# Autodesk Inventor assembly: Segment_Traeger_v1
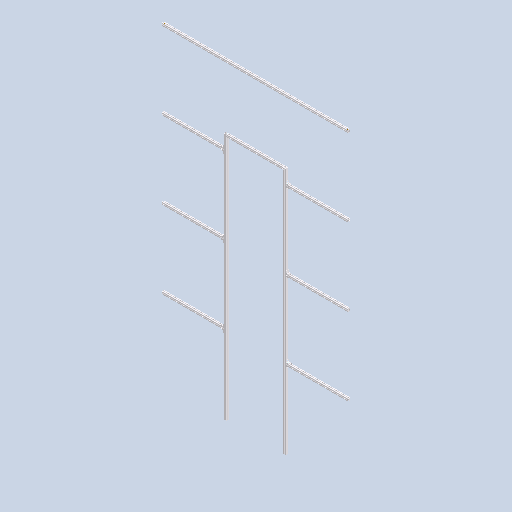
[picture p0: Inventor's stored thumbnail of the model, 512x512]
Saved by Autodesk Inventor 2025.1 (Build 291241000, 241)
## iProperties
Created: 2024-10-13
Part Number: Segment_Traeger_v1
Document SubType Name: Assembly
Designer: Kai Altwicker
Author: Kai Altwicker
## Documents named in this file (8)
- C:\Users\tallA\Repos\VolumanXR\hardware-capture\cad\rig_v1\Segment_Traeger_Tuer_v1.iam
- C:\Users\tallA\Repos\VolumanXR\hardware-capture\cad\rig_v1\Profil_5_20x20_1500.ipt
- C:\Users\tallA\Repos\VolumanXR\hardware-capture\cad\rig_v1\Profil_5_20x20_500.ipt
- C:\Users\tallA\Repos\VolumanXR\hardware-capture\cad\rig_v1\Profil_5_20x20_2000.ipt
- C:\Users\tallA\Repos\VolumanXR\hardware-capture\cad\rig_v1\Profil_5_20x20_460.ipt
- C:\Users\tallA\Repos\VolumanXR\hardware-capture\cad\Library\Zentrierplattensatz_5\Zentrierplattensatz_5\Zentrierplattensatz_5.ipt
- C:\Users\tallA\Repos\VolumanXR\hardware-capture\cad\Library\Winkelsatz_20x20_einfach\Winkelsatz_20x20_einfach\Winkelsatz_20x20_einfach.ipt
- C:\Users\tallA\Repos\VolumanXR\hardware-capture\cad\dimensions.xlsx
## Components (24 placed, 6 different names)
1. Profil_5_20x20_1500:2 — Passend:1, Passend:2, Passend:3, Fluchtend:1, Fluchtend:2, Passend:4, Fluchtend:6
2. Profil_5_20x20_2000:1 — Passend:5, Fluchtend:5, Fluchtend:6, Passend:10, Fluchtend:10, Fluchtend:11, Fluchtend:12, Passend:13, Passend:15
3. Profil_5_20x20_2000:2 — Passend:7, Passend:11, Fluchtend:12, Fluchtend:13, Passend:12, Passend:17, Passend:18
4. Profil_5_20x20_460:1 — Passend:8, Passend:9, Fluchtend:8, Fluchtend:9, Fluchtend:10, Fluchtend:11, Passend:12
5. Zentrierplattensatz_5:1 — Passend:9, Fluchtend:8, Passend:11
6. Zentrierplattensatz_5:2 — Passend:8, Fluchtend:9, Passend:10
7. Profil_5_20x20_500:2 — Passend:4, Fluchtend:3, Fluchtend:4, Passend:7, Fluchtend:13, Passend:19, Fluchtend:16, Passend:20, Fluchtend:17
8. Profil_5_20x20_500:1 — Passend:3, Fluchtend:1, Fluchtend:2, Fluchtend:3, Fluchtend:4, Passend:5, Fluchtend:5, Fluchtend:14, Passend:14, Passend:16, Fluchtend:15
9. Profil_5_20x20_500:3
10. Profil_5_20x20_500:4
11. Profil_5_20x20_500:5
12. Profil_5_20x20_500:6
13. Winkelsatz_20x20_einfach:3 — Passend:17, Passend:20, Fluchtend:17
14. Winkelsatz_20x20_einfach:4 — Passend:18, Passend:19, Fluchtend:16
15. Winkelsatz_20x20_einfach:2 — Passend:15, Passend:16, Fluchtend:15
16. Winkelsatz_20x20_einfach:1 — Passend:13, Fluchtend:14, Passend:14
17. Winkelsatz_20x20_einfach:5
18. Winkelsatz_20x20_einfach:6
19. Winkelsatz_20x20_einfach:7
20. Winkelsatz_20x20_einfach:8
21. Winkelsatz_20x20_einfach:9
22. Winkelsatz_20x20_einfach:10
23. Winkelsatz_20x20_einfach:11
24. Winkelsatz_20x20_einfach:12
## Component patterns: (3 elements, first: Profil_5_20x20_500:2 + Profil_5_20x20_500:1), (3 elements, first: Winkelsatz_20x20_einfach:3 + Winkelsatz_20x20_einfach:4 + Winkelsatz_20x20_einfach:2 + Winkelsatz_20x20_einfach:1)
## Relationships (35: Mate 19, Flush 16)
- Passend:1 [Mate]: Profil_5_20x20_1500:2
- Passend:2 [Mate]: Profil_5_20x20_1500:2
- Passend:3 [Mate]: Profil_5_20x20_1500:2 ↔ Profil_5_20x20_500:1
- Fluchtend:1 [Flush] (625 mm): Profil_5_20x20_1500:2 ↔ Profil_5_20x20_500:1
- Fluchtend:2 [Flush]: Profil_5_20x20_1500:2 ↔ Profil_5_20x20_500:1
- Passend:4 [Mate]: Profil_5_20x20_1500:2 ↔ Profil_5_20x20_500:2
- Fluchtend:3 [Flush]: Profil_5_20x20_500:2 ↔ Profil_5_20x20_500:1
- Fluchtend:4 [Flush]: Profil_5_20x20_500:2 ↔ Profil_5_20x20_500:1
- Passend:5 [Mate]: Profil_5_20x20_2000:1 ↔ Profil_5_20x20_500:1
- Fluchtend:5 [Flush]: Profil_5_20x20_2000:1 ↔ Profil_5_20x20_500:1
- Fluchtend:6 [Flush] (-2500 mm): Profil_5_20x20_1500:2 ↔ Profil_5_20x20_2000:1
- Passend:7 [Mate]: Profil_5_20x20_2000:2 ↔ Profil_5_20x20_500:2
- Passend:8 [Mate]: Profil_5_20x20_460:1 ↔ Zentrierplattensatz_5:2
- Passend:9 [Mate]: Profil_5_20x20_460:1 ↔ Zentrierplattensatz_5:1
- Fluchtend:8 [Flush] (0.5 mm): Profil_5_20x20_460:1 ↔ Zentrierplattensatz_5:1
- Fluchtend:9 [Flush] (0.5 mm): Profil_5_20x20_460:1 ↔ Zentrierplattensatz_5:2
- Passend:10 [Mate]: Profil_5_20x20_2000:1 ↔ Zentrierplattensatz_5:2
- Fluchtend:10 [Flush]: Profil_5_20x20_2000:1 ↔ Profil_5_20x20_460:1
- Fluchtend:11 [Flush] (-1.375 mm): Profil_5_20x20_2000:1 ↔ Profil_5_20x20_460:1
- Passend:11 [Mate]: Profil_5_20x20_2000:2 ↔ Zentrierplattensatz_5:1
- Fluchtend:12 [Flush]: Profil_5_20x20_2000:1 ↔ Profil_5_20x20_2000:2
- Fluchtend:13 [Flush]: Profil_5_20x20_2000:2 ↔ Profil_5_20x20_500:2
- Passend:12 [Mate]: Profil_5_20x20_2000:2 ↔ Profil_5_20x20_460:1
- Passend:13 [Mate]: Profil_5_20x20_2000:1 ↔ Winkelsatz_20x20_einfach:1
- Fluchtend:14 [Flush]: Profil_5_20x20_500:1 ↔ Winkelsatz_20x20_einfach:1
- Passend:14 [Mate]: Profil_5_20x20_500:1 ↔ Winkelsatz_20x20_einfach:1
- Passend:15 [Mate]: Profil_5_20x20_2000:1 ↔ Winkelsatz_20x20_einfach:2
- Passend:16 [Mate]: Profil_5_20x20_500:1 ↔ Winkelsatz_20x20_einfach:2
- Fluchtend:15 [Flush]: Profil_5_20x20_500:1 ↔ Winkelsatz_20x20_einfach:2
- Passend:17 [Mate]: Profil_5_20x20_2000:2 ↔ Winkelsatz_20x20_einfach:3
- Passend:18 [Mate]: Profil_5_20x20_2000:2 ↔ Winkelsatz_20x20_einfach:4
- Passend:19 [Mate]: Profil_5_20x20_500:2 ↔ Winkelsatz_20x20_einfach:4
- Fluchtend:16 [Flush]: Profil_5_20x20_500:2 ↔ Winkelsatz_20x20_einfach:4
- Passend:20 [Mate]: Profil_5_20x20_500:2 ↔ Winkelsatz_20x20_einfach:3
- Fluchtend:17 [Flush]: Profil_5_20x20_500:2 ↔ Winkelsatz_20x20_einfach:3
## Named parameters: d_tol = 0.3 mm, d_wand = 1.5 mm, d_traeger = 625 mm, l_profil_40x40 = 2500 mm, h_profil_40x40 = 40 mm, h_profil_20x20 = 20 mm, b_profil_40x40 = 40 mm, b_profil_20x20 = 20 mm, l_profil_20x20 = 1500 mm, D_oct = 3621.32034 mm, D_dode = 8196.15242 mm, D_hexadeca = 7541.00924 mm
